# Autodesk Inventor assembly: right pneumatics board
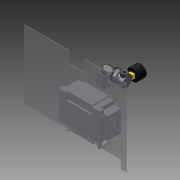
[picture p0: Inventor's stored thumbnail of the model, 180x180]
Saved by Autodesk Inventor 2014 (Build 180170000, 170)
## iProperties
Created: 2014-01-20
Part Number: right pneumatics board
Document SubType Name: Assembly
Designer: Arpan
Author: Arpan
## Documents named in this file (4)
- C:\Users\Andrew Toennies\Documents\GitHub\2014buildCAD\pneumatics board\right pneumatics board.iam
- C:\Users\Andrew Toennies\Documents\GitHub\2014buildCAD\pneumatics board\pneumatics board 1.ipt
- C:\Users\Andrew Toennies\Documents\GitHub\2014buildCAD\pneumatics board\pneumatics thing 2.iam
- C:\Users\Andrew Toennies\Documents\GitHub\2014buildCAD\New Shooter\Manifold and Valves\Manifold.iam
## Components (3 placed, 3 different names)
1. pneumatics board 1:1 — Mate:1, Mate:2, Flush:1, Flush:2
2. pneumatics thing 2:1 [sub-assembly] — Mate:1
3. Manifold:1 [sub-assembly] — Mate:2, Flush:1, Flush:2
## Relationships (4: Mate 2, Flush 2)
- Mate:1: pneumatics board 1:1 ↔ pneumatics thing 2:1
- Mate:2: pneumatics board 1:1 ↔ Manifold:1
- Flush:1 (-76.2 mm): pneumatics board 1:1 ↔ Manifold:1
- Flush:2 (127 mm): pneumatics board 1:1 ↔ Manifold:1
